# Autodesk Inventor assembly: ADSK-MH-10028
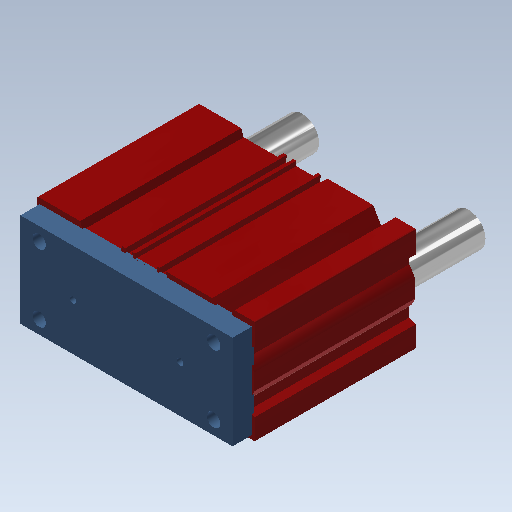
[picture p0: Inventor's stored thumbnail of the model, 512x512]
Saved by Autodesk Inventor 2020.2 (Build 242310000, 310)
## iProperties
Created: 2013-08-01
Part Number: ADSK-MH-10028
Document SubType Name: Assembly
Designer: Demir Ali
Description: Pneumatic Cylinder
Engineer: Demir Ali
Checked By: Demir Ali
Company: Autodesk Ltd
Author: Demir Ali
Keywords: Roller Conveyor
Revision Number: A
## Documents named in this file (3)
- C:\Users\peter\source\repos\InventorDA-FLC\Dataset\Discharge Conveyor\ADSK-MH-10028.iam
- C:\Users\peter\source\repos\InventorDA-FLC\Dataset\Discharge Conveyor\ADSK-MH-10029.ipt
- C:\Users\peter\source\repos\InventorDA-FLC\Dataset\Discharge Conveyor\ADSK-MH-10030.ipt
## Components (2 placed, 2 different names)
1. ADSK-MH-10029:1 — Mate:1, Mate:2, Mate:3
2. ADSK-MH-10030:1 — Mate:1, Mate:2, Mate:3
## Relationships (3: Mate 3)
- Mate:1: ADSK-MH-10029:1 ↔ ADSK-MH-10030:1
- Mate:2: ADSK-MH-10029:1 ↔ ADSK-MH-10030:1
- Mate:3: ADSK-MH-10029:1 ↔ ADSK-MH-10030:1
